# Autodesk Inventor assembly: SLIM_ASSEMBLED
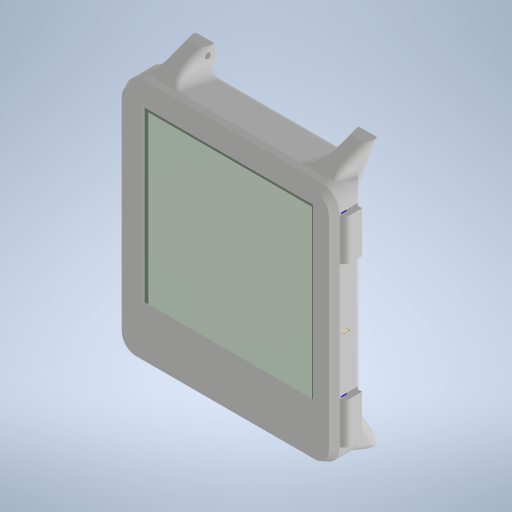
[picture p0: Inventor's stored thumbnail of the model, 512x512]
Saved by Autodesk Inventor 2023 (Build 270158000, 158)
## iProperties
Created: 2021-08-24
Part Number: SLIM_ASSEMBLED
Document SubType Name: Assembly
Designer: nigel
Author: nigel
## Documents named in this file (6)
- D:\NIGEL\Documents\GitHub\Watchy-CAD\CAD\Cases\SlimV5\SLIM_ASSEMBLED_V5.iam
- D:\NIGEL\Documents\GitHub\Watchy-CAD\CAD\Base Model\WATCHY_CUT.iam
- D:\NIGEL\Documents\GitHub\Watchy-CAD\CAD\Base Model\Battery_402535.ipt
- D:\NIGEL\Documents\GitHub\Watchy-CAD\CAD\Cases\SlimV5\Bottom_V5.ipt
- D:\NIGEL\Documents\GitHub\Watchy-CAD\CAD\Cases\SlimV5\Top_V5.ipt
- D:\NIGEL\Documents\GitHub\Watchy-CAD\CAD\Cases\SlimV5\WatchyCaseParams.xlsx
## Components (4 placed, 4 different names)
1. Bottom_V5:1
2. WATCHY_CUT:1 [sub-assembly] — Mate:9
3. Top_V5:1
4. Battery_402535:1 — Mate:9
## Relationships (7: Flush 4, Mate 3)
- [Flush]: Bottom_V5:1 ↔ WATCHY_CUT:1
- [Flush]: Bottom_V5:1 ↔ WATCHY_CUT:1
- [Flush]: Bottom_V5:1 ↔ Top_V5:1
- [Mate]: Bottom_V5:1 ↔ Top_V5:1
- [Mate]: Bottom_V5:1 ↔ WATCHY_CUT:1
- [Flush]: Bottom_V5:1 ↔ Top_V5:1
- Mate:9: WATCHY_CUT:1 ↔ Battery_402535:1
## Named parameters: pcb_thickness = 0.94 mm, case_thickness = 1 mm, electronics_thickness = 7 mm, usb_height = 4 mm, strap_pin_depth = 2.3 mm, top_thickness = 0.2 mm, display_thickness = 1.2 mm
